# Autodesk Inventor assembly: SC-0-02-Geneva Assembly 12
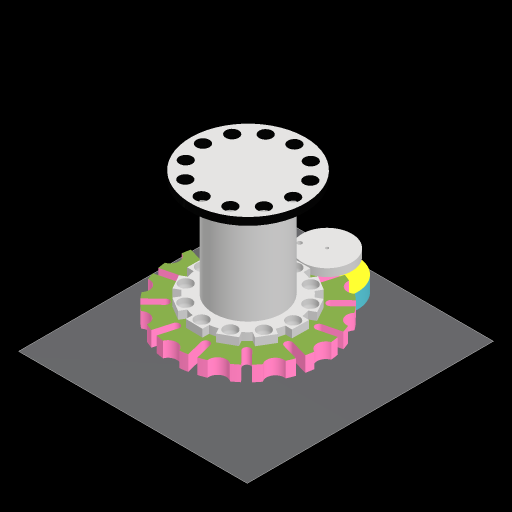
[picture p0: Inventor's stored thumbnail of the model, 512x512]
Saved by Autodesk Inventor 2023 (Build 270158000, 158)
## iProperties
Created: 2022-10-22
Part Number: SC-0-02-Geneva Assembly 12
Document SubType Name: Assembly
Designer: annah
Author: annah
## Documents named in this file (6)
- C:\Users\annah\Desktop\inventor\SC-0-02-Geneva Assembly 12.iam
- C:\Users\annah\Desktop\inventor\SC-1-01-Bridge.ipt
- C:\Users\annah\Desktop\inventor\SC-1-02-Geneva Circle Arc.ipt
- C:\Users\annah\Desktop\inventor\SC-1-01-Geneva Gear 12.ipt
- C:\Users\annah\Desktop\inventor\SC-1-01-Test Tube Rack.ipt
- C:\Users\annah\Desktop\inventor\SC-1-01-Circle Arc Cover.ipt
## Components (5 placed, 5 different names)
1. SC-1-01-Bridge:1 — Mate:1, Mate:2, Mate:3, Mate:4, Mate:5
2. SC-1-02-Geneva Circle Arc:1 — Mate:2, Mate:3, Mate:8, Mate:9, Mate:10
3. SC-1-01-Geneva Gear 12:1 — Mate:4, Mate:5, Rigid:1
4. SC-1-01-Test Tube Rack:1 — Rigid:1
5. SC-1-01-Circle Arc Cover:1 — Mate:8, Mate:9, Mate:10
## Relationships (9: Mate 8, WeldJoint 1)
- Mate:1: SC-1-01-Bridge:1
- Mate:2: SC-1-01-Bridge:1 ↔ SC-1-02-Geneva Circle Arc:1
- Mate:3: SC-1-01-Bridge:1 ↔ SC-1-02-Geneva Circle Arc:1
- Mate:4: SC-1-01-Bridge:1 ↔ SC-1-01-Geneva Gear 12:1
- Mate:5: SC-1-01-Bridge:1 ↔ SC-1-01-Geneva Gear 12:1
- Mate:8: SC-1-02-Geneva Circle Arc:1 ↔ SC-1-01-Circle Arc Cover:1
- Mate:9: SC-1-02-Geneva Circle Arc:1 ↔ SC-1-01-Circle Arc Cover:1
- Mate:10: SC-1-02-Geneva Circle Arc:1 ↔ SC-1-01-Circle Arc Cover:1
- Rigid:1 [WeldJoint]: SC-1-01-Geneva Gear 12:1 ↔ SC-1-01-Test Tube Rack:1
